# Autodesk Inventor assembly: 힘-토크 측정기기
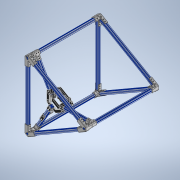
[picture p0: Inventor's stored thumbnail of the model, 180x180]
Saved by Autodesk Inventor 2021 (Build 250183000, 183)
## iProperties
Created: 2021-01-21
Part Number: 힘-토크 측정기기
Document SubType Name: Assembly
Designer: leejun
Author: leejun
## Documents named in this file (21)
- C:\Users\leejun\Desktop\EE495\force_thrust_meter\cad\v2\힘-토크 측정기기_v2.iam
- C:\Users\leejun\Desktop\EE495\force_thrust_meter\cad\v2\[한진데이타]_4선식_저가형_로드셀_5Kg.ipt
- C:\Users\leejun\Desktop\EE495\force_thrust_meter\cad\v2\motor_mount_v2.ipt
- C:\Users\leejun\Desktop\EE495\force_thrust_meter\cad\v2\bldc_sample\BLDC motor\BLDC motor.iam
- C:\Users\leejun\Desktop\EE495\force_thrust_meter\cad\v2\base_v2.ipt
- C:\Users\leejun\Desktop\EE495\force_thrust_meter\cad\v2\connector_v2.ipt
- C:\Users\leejun\Desktop\EE495\force_thrust_meter\cad\v2\motor_mount.ipt
- C:\Users\leejun\Desktop\EE495\force_thrust_meter\cad\v2\torque_base.ipt
- C:\Users\leejun\Desktop\EE495\force_thrust_meter\cad\v2\profile_bracket.ipt
- C:\Users\leejun\Desktop\EE495\force_thrust_meter\cad\v2\300mm 2020.ipt
- C:\Users\leejun\Desktop\EE495\force_thrust_meter\cad\v2\600mm 2020.ipt
- C:\Users\leejun\Desktop\EE495\force_thrust_meter\cad\v2\case_corner.ipt
- C:\Users\leejun\Desktop\EE495\force_thrust_meter\cad\v2\500mm 2020.ipt
- C:\Users\leejun\Desktop\EE495\force_thrust_meter\cad\v2\torque_calibrator.ipt
- C:\Users\leejun\Desktop\EE495\force_thrust_meter\cad\v2\pully_holder.ipt
- C:\Users\jun85\Desktop\개별연구\힘-토크 측정기기_v2\힘-토크 측정기기\AIP\FEA\dhwt064ps.fins
- C:\Users\jun85\Desktop\개별연구\힘-토크 측정기기_v2\힘-토크 측정기기\AIP\FEA\dhwt064ps.fsat
- C:\Users\jun85\Desktop\개별연구\힘-토크 측정기기_v2\힘-토크 측정기기\AIP\FEA\dhwt064ps.ftes
- C:\Users\jun85\Desktop\개별연구\힘-토크 측정기기_v2\힘-토크 측정기기\AIP\FEA\dhwt064ps.fwiz
- C:\Users\jun85\Desktop\개별연구\힘-토크 측정기기_v2\힘-토크 측정기기\AIP\FEA\dhwt064tc.fmsh
- C:\Users\jun85\Desktop\개별연구\힘-토크 측정기기_v2\힘-토크 측정기기\AIP\FEA\dhwt064td.fres
## Components (35 placed, 14 different names)
1. [한진데이타]_4선식_저가형_로드셀_5Kg:1 — 메이트:48, 메이트:50, 플러쉬:5, 메이트:65, 메이트:66, 메이트:67
2. motor_mount_v2:1 — 플러쉬:1, 플러쉬:2, 플러쉬:3, 메이트:48, 메이트:49, 메이트:50, 메이트:51, 메이트:52, 메이트:53, 메이트:58, 플러쉬:4, 플러쉬:5, 메이트:87, 메이트:88, 메이트:89
3. [한진데이타]_4선식_저가형_로드셀_5Kg:2 — 메이트:27, 메이트:28, 메이트:30
4. [한진데이타]_4선식_저가형_로드셀_5Kg:3 — 메이트:49, 메이트:58, 플러쉬:4, 메이트:59, 메이트:60, 메이트:61
5. [한진데이타]_4선식_저가형_로드셀_5Kg:4 — 메이트:22, 메이트:23, 메이트:24, 메이트:40, 메이트:41, 메이트:42
6. [한진데이타]_4선식_저가형_로드셀_5Kg:5 — 메이트:25, 메이트:26, 메이트:29
7. BLDC motor:1 [sub-assembly] — 메이트:54, 접선:1, 접선:2, 접선:3
8. motor_mount:1 — 메이트:51, 메이트:52, 메이트:53, 메이트:54, 접선:1, 접선:2, 접선:3
9. base_v2:1 — 메이트:22, 메이트:23, 메이트:24, 메이트:25, 메이트:26, 메이트:27, 메이트:28, 메이트:29, 메이트:30, 메이트:68, 메이트:69, 플러쉬:6
10. connector_v2:1 — 메이트:40, 메이트:41, 메이트:42, 메이트:62, 메이트:63, 메이트:64
11. torque_base:1 — 메이트:65, 메이트:66, 메이트:67
12. torque_base:2 — 메이트:59, 메이트:60, 메이트:61, 메이트:62, 메이트:63, 메이트:64
13. torque_calibrator:1 — 메이트:87, 메이트:88, 메이트:89
14. pully_holder:1 — 메이트:90, 메이트:91
15. 600mm 2020:1 — 메이트:73, 메이트:74, 메이트:75, 메이트:76, 메이트:77, 메이트:84, 메이트:85, 메이트:86
16. 500mm 2020:2
17. case_corner:2 — 메이트:84, 메이트:85, 메이트:86, 메이트:92
18. 500mm 2020:1 — 메이트:78, 메이트:79, 메이트:80
19. case_corner:1 — 메이트:75, 메이트:76, 메이트:77, 메이트:78, 메이트:79, 메이트:80, 메이트:93
20. 300mm 2020:1 — 메이트:68, 메이트:69, 메이트:70, 메이트:71, 메이트:72, 플러쉬:6
21. profile_bracket:1 — 메이트:70, 메이트:71, 메이트:72, 메이트:73, 메이트:74, 메이트:92, 메이트:93
22. 600mm 2020:2
23. 500mm 2020:3
24. case_corner:3
25. 500mm 2020:4
26. case_corner:4
27. 300mm 2020:2
28. profile_bracket:2
29. 600mm 2020:3
30. 500mm 2020:5
31. case_corner:5
32. 500mm 2020:6
33. case_corner:6
34. 300mm 2020:3 — 메이트:90, 메이트:91
35. profile_bracket:3
## Component patterns: (3 elements, first: 600mm 2020:1 + 500mm 2020:2 + case_corner:2 + 500mm 2020:1 + case_corner:1 + 300mm 2020:1 + profile_bracket:1)
## Relationships (64: Mate 55, Flush 6, Tangent 3)
- 플러쉬:1 [Flush]: motor_mount_v2:1
- 플러쉬:2 [Flush]: motor_mount_v2:1
- 플러쉬:3 [Flush]: motor_mount_v2:1
- 메이트:22 [Mate]: [한진데이타]_4선식_저가형_로드셀_5Kg:4 ↔ base_v2:1
- 메이트:23 [Mate]: [한진데이타]_4선식_저가형_로드셀_5Kg:4 ↔ base_v2:1
- 메이트:24 [Mate]: [한진데이타]_4선식_저가형_로드셀_5Kg:4 ↔ base_v2:1
- 메이트:25 [Mate]: [한진데이타]_4선식_저가형_로드셀_5Kg:5 ↔ base_v2:1
- 메이트:26 [Mate]: [한진데이타]_4선식_저가형_로드셀_5Kg:5 ↔ base_v2:1
- 메이트:27 [Mate]: [한진데이타]_4선식_저가형_로드셀_5Kg:2 ↔ base_v2:1
- 메이트:28 [Mate]: [한진데이타]_4선식_저가형_로드셀_5Kg:2 ↔ base_v2:1
- 메이트:29 [Mate]: [한진데이타]_4선식_저가형_로드셀_5Kg:5 ↔ base_v2:1
- 메이트:30 [Mate]: [한진데이타]_4선식_저가형_로드셀_5Kg:2 ↔ base_v2:1
- 메이트:40 [Mate]: [한진데이타]_4선식_저가형_로드셀_5Kg:4 ↔ connector_v2:1
- 메이트:41 [Mate]: [한진데이타]_4선식_저가형_로드셀_5Kg:4 ↔ connector_v2:1
- 메이트:42 [Mate]: [한진데이타]_4선식_저가형_로드셀_5Kg:4 ↔ connector_v2:1
- 메이트:48 [Mate]: [한진데이타]_4선식_저가형_로드셀_5Kg:1 ↔ motor_mount_v2:1
- 메이트:49 [Mate]: motor_mount_v2:1 ↔ [한진데이타]_4선식_저가형_로드셀_5Kg:3
- 메이트:50 [Mate]: [한진데이타]_4선식_저가형_로드셀_5Kg:1 ↔ motor_mount_v2:1
- 메이트:51 [Mate]: motor_mount_v2:1 ↔ motor_mount:1
- 메이트:52 [Mate]: motor_mount_v2:1 ↔ motor_mount:1
- 메이트:53 [Mate]: motor_mount_v2:1 ↔ motor_mount:1
- 메이트:54 [Mate]: BLDC motor:1 ↔ motor_mount:1
- 접선:1 [Tangent] (0.1 mm): BLDC motor:1 ↔ motor_mount:1
- 접선:2 [Tangent] (0.1 mm): BLDC motor:1 ↔ motor_mount:1
- 접선:3 [Tangent] (0.1 mm): BLDC motor:1 ↔ motor_mount:1
- 메이트:58 [Mate]: motor_mount_v2:1 ↔ [한진데이타]_4선식_저가형_로드셀_5Kg:3
- 플러쉬:4 [Flush]: motor_mount_v2:1 ↔ [한진데이타]_4선식_저가형_로드셀_5Kg:3
- 플러쉬:5 [Flush]: [한진데이타]_4선식_저가형_로드셀_5Kg:1 ↔ motor_mount_v2:1
- 메이트:59 [Mate]: [한진데이타]_4선식_저가형_로드셀_5Kg:3 ↔ torque_base:2
- 메이트:60 [Mate]: [한진데이타]_4선식_저가형_로드셀_5Kg:3 ↔ torque_base:2
- 메이트:61 [Mate]: [한진데이타]_4선식_저가형_로드셀_5Kg:3 ↔ torque_base:2
- 메이트:62 [Mate]: connector_v2:1 ↔ torque_base:2
- 메이트:63 [Mate]: connector_v2:1 ↔ torque_base:2
- 메이트:64 [Mate]: connector_v2:1 ↔ torque_base:2
- 메이트:65 [Mate]: [한진데이타]_4선식_저가형_로드셀_5Kg:1 ↔ torque_base:1
- 메이트:66 [Mate]: [한진데이타]_4선식_저가형_로드셀_5Kg:1 ↔ torque_base:1
- 메이트:67 [Mate]: [한진데이타]_4선식_저가형_로드셀_5Kg:1 ↔ torque_base:1
- 메이트:68 [Mate] (0.5 mm): base_v2:1 ↔ 300mm 2020:1
- 메이트:69 [Mate] (0.5 mm): base_v2:1 ↔ 300mm 2020:1
- 메이트:70 [Mate] (0.5 mm): 300mm 2020:1 ↔ profile_bracket:1
- 메이트:71 [Mate] (0.5 mm): 300mm 2020:1 ↔ profile_bracket:1
- 메이트:72 [Mate]: 300mm 2020:1 ↔ profile_bracket:1
- 메이트:73 [Mate] (0.5 mm): 600mm 2020:1 ↔ profile_bracket:1
- 메이트:74 [Mate] (0.5 mm): 600mm 2020:1 ↔ profile_bracket:1
- 메이트:75 [Mate] (0.5 mm): 600mm 2020:1 ↔ case_corner:1
- 메이트:76 [Mate] (0.5 mm): 600mm 2020:1 ↔ case_corner:1
- 메이트:77 [Mate]: 600mm 2020:1 ↔ case_corner:1
- 메이트:78 [Mate]: 500mm 2020:1 ↔ case_corner:1
- 메이트:79 [Mate] (0.5 mm): 500mm 2020:1 ↔ case_corner:1
- 메이트:80 [Mate] (0.5 mm): 500mm 2020:1 ↔ case_corner:1
- [Mate]: 500mm 2020:2 ↔ case_corner:2
- [Mate] (0.5 mm): 500mm 2020:2 ↔ case_corner:2
- [Mate] (0.5 mm): 500mm 2020:2 ↔ case_corner:2
- 메이트:84 [Mate] (0.5 mm): 600mm 2020:1 ↔ case_corner:2
- 메이트:85 [Mate]: 600mm 2020:1 ↔ case_corner:2
- 메이트:86 [Mate] (0.5 mm): 600mm 2020:1 ↔ case_corner:2
- 메이트:87 [Mate]: motor_mount_v2:1 ↔ torque_calibrator:1
- 메이트:88 [Mate]: motor_mount_v2:1 ↔ torque_calibrator:1
- 메이트:89 [Mate]: motor_mount_v2:1 ↔ torque_calibrator:1
- 메이트:90 [Mate] (0.5 mm): pully_holder:1 ↔ 300mm 2020:3
- 메이트:91 [Mate] (0.5 mm): pully_holder:1 ↔ 300mm 2020:3
- 플러쉬:6 [Flush] (-3 mm): base_v2:1 ↔ 300mm 2020:1
- 메이트:92 [Mate] (400 mm): case_corner:2 ↔ profile_bracket:1
- 메이트:93 [Mate]: case_corner:1 ↔ profile_bracket:1
## Named parameters: sa_0 = 170, d114_d111 = 0 mm, d115_d112 = 0.5 mm, d116_d113 = 0.5 mm
note: some values were not read from the file. Shown as the stored number, unit unknown: "sa_0".
